# Autodesk Inventor assembly: norm bottle
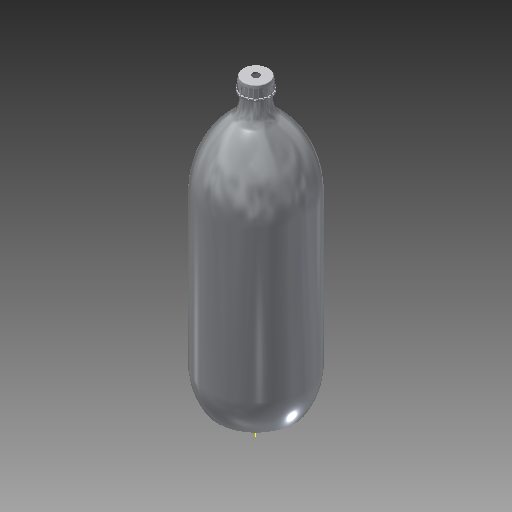
[picture p0: Inventor's stored thumbnail of the model, 512x512]
Saved by Autodesk Inventor 2019 (Build 230136000, 136)
## iProperties
Created: 2015-04-14
Part Number: norm bottle
Document SubType Name: Assembly
Designer: Colin
Author: Colin
## Documents named in this file (3)
- D:\Ian\Documents\Projects\autoturret\mechanical design\norm bottle.iam
- D:\Ian\Documents\Projects\autoturret\mechanical design\bottle.ipt
- D:\Ian\Documents\Projects\autoturret\mechanical design\cap.ipt
## Components (2 placed, 2 different names)
1. bottle:1 — Mate:1, Mate:2
2. cap:1 — Mate:1, Mate:3
## Relationships (4: Mate 4)
- Mate:1: bottle:1 ↔ cap:1
- Mate:2: bottle:1
- Mate:3: cap:1
- Mate:4
